# Autodesk Inventor assembly: FullElevator
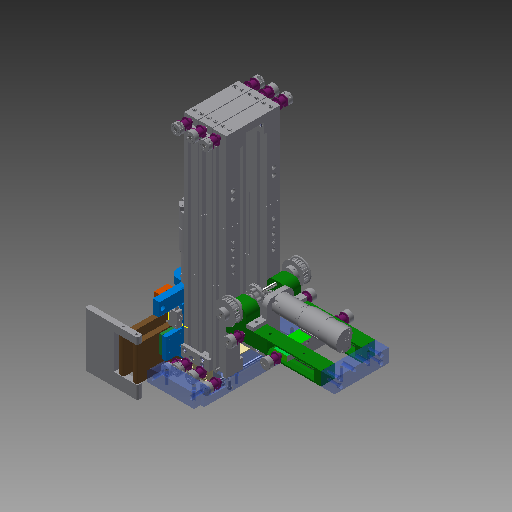
[picture p0: Inventor's stored thumbnail of the model, 512x512]
Saved by Autodesk Inventor 2019 (Build 230136000, 136)
## iProperties
Created: 2019-09-28
Part Number: FullElevator
Document SubType Name: Assembly
Designer: james
Author: james
## Documents named in this file (15)
- F:\JimsDesign\Jims2020FTC\FullElevator.iam
- F:\JimsDesign\Jims2020FTC\ElevBackFrame.iam
- F:\JimsDesign\Jims2020FTC\EvelMidFrame.iam
- F:\JimsDesign\Jims2020FTC\EvelFrontFrame.iam
- F:\JimsDesign\Jims2020FTC\Carrier.iam
- F:\JimsDesign\Jims2020FTC\BackTopBeams.ipt
- F:\JimsDesign\Jims2020FTC\FullElevatorShart.iam
- F:\JimsDesign\Jims2020FTC\ElevDriveShaft.iam
- F:\JimsDesign\Library\ServoCity\5202-0002-0071 part.ipt
- F:\JimsDesign\Library\ServoCity\545548 assembly.iam
- F:\JimsDesign\Library\ServoCity\615460.ipt
- F:\JimsDesign\Library\ServoCity\615456 assembly.iam
- F:\JimsDesign\Jims2020FTC\SliderSlider.ipt
- F:\JimsDesign\Jims2020FTC\BackEndSlider.ipt
- F:\JimsDesign\Jims2020FTC\SliderMotorMount.ipt
## Components (16 placed, 14 different names)
1. ElevBackFrame:1 [sub-assembly] — Mate:32, Mate:33, Mate:34, Flush:7, Mate:54, Mate:55
2. EvelMidFrame:1 [sub-assembly] — Mate:54, Mate:55, Mate:56, Mate:57
3. EvelFrontFrame:1 [sub-assembly] — Mate:56, Mate:57, Mate:58, Mate:59
4. BackTopBeams:1 — Flush:4, Mate:23, Mate:25, Mate:32, Mate:33, Mate:34, Flush:5, Flush:6, Mate:35, Mate:36, Mate:37, Mate:46, Mate:49, Mate:50
5. BackTopBeams:2 — Flush:4, Flush:5, Flush:6, Flush:7, Mate:44, Mate:45, Mate:51
6. FullElevatorShart:1 [sub-assembly] — Mate:25, Mate:37
7. FullElevatorShart:3 [sub-assembly] — Mate:23, Mate:47
8. ElevDriveShaft:1 [sub-assembly] — Mate:35, Mate:36, Mate:40, Mate:41
9. 5202-0002-0071 part:1 — Mate:42, Flush:8, Mate:52, Mate:53
10. Carrier:1 [sub-assembly] — Mate:58, Mate:59
11. 545548 assembly:1 [sub-assembly] — Mate:38, Mate:40
12. 615460:1 — Mate:38, Mate:41
13. 615456 assembly:1 [sub-assembly] — Mate:42, Flush:8
14. SliderSlider:1 — Mate:47, Mate:48
15. BackEndSlider:1 — Mate:44, Mate:45, Mate:46, Mate:48
16. SliderMotorMount:1 — Mate:49, Mate:50, Mate:51, Mate:52, Mate:53
## Relationships (33: Mate 28, Flush 5)
- Flush:4: BackTopBeams:1 ↔ BackTopBeams:2
- Mate:23: BackTopBeams:1 ↔ FullElevatorShart:3
- Mate:25: BackTopBeams:1 ↔ FullElevatorShart:1
- Mate:32: ElevBackFrame:1 ↔ BackTopBeams:1
- Mate:33: ElevBackFrame:1 ↔ BackTopBeams:1
- Mate:34: ElevBackFrame:1 ↔ BackTopBeams:1
- Flush:5: BackTopBeams:1 ↔ BackTopBeams:2
- Flush:6: BackTopBeams:1 ↔ BackTopBeams:2
- Mate:35: BackTopBeams:1 ↔ ElevDriveShaft:1
- Mate:36: BackTopBeams:1 ↔ ElevDriveShaft:1
- Flush:7: ElevBackFrame:1 ↔ BackTopBeams:2
- Mate:37: BackTopBeams:1 ↔ FullElevatorShart:1
- Mate:38: 545548 assembly:1 ↔ 615460:1
- Mate:40: ElevDriveShaft:1 ↔ 545548 assembly:1
- Mate:41: ElevDriveShaft:1 ↔ 615460:1
- Mate:42: 5202-0002-0071 part:1 ↔ 615456 assembly:1
- Flush:8: 5202-0002-0071 part:1 ↔ 615456 assembly:1
- Mate:44: BackTopBeams:2 ↔ BackEndSlider:1
- Mate:45: BackTopBeams:2 ↔ BackEndSlider:1
- Mate:46: BackTopBeams:1 ↔ BackEndSlider:1
- Mate:47: FullElevatorShart:3 ↔ SliderSlider:1
- Mate:48: SliderSlider:1 ↔ BackEndSlider:1
- Mate:49: BackTopBeams:1 ↔ SliderMotorMount:1
- Mate:50: BackTopBeams:1 ↔ SliderMotorMount:1
- Mate:51: BackTopBeams:2 ↔ SliderMotorMount:1
- Mate:52: 5202-0002-0071 part:1 ↔ SliderMotorMount:1
- Mate:53: 5202-0002-0071 part:1 ↔ SliderMotorMount:1
- Mate:54: ElevBackFrame:1 ↔ EvelMidFrame:1
- Mate:55: ElevBackFrame:1 ↔ EvelMidFrame:1
- Mate:56: EvelMidFrame:1 ↔ EvelFrontFrame:1
- Mate:57: EvelMidFrame:1 ↔ EvelFrontFrame:1
- Mate:58: EvelFrontFrame:1 ↔ Carrier:1
- Mate:59: EvelFrontFrame:1 ↔ Carrier:1
